# Autodesk Inventor assembly: uchwytDoSzyny
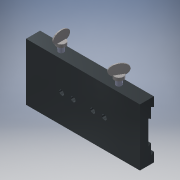
[picture p0: Inventor's stored thumbnail of the model, 180x180]
Saved by Autodesk Inventor 2019 (Build 230136000, 136)
## iProperties
Created: 2020-08-30
Part Number: uchwytDoSzyny
Document SubType Name: Assembly
Designer: estee
Author: estee
## Documents named in this file (3)
- C:\Users\estee\OneDrive\Pulpit\estere\1\MUM\najnowszyGIT\Mechanika\Moduł obrotu RET Estera\projejt\projejt\uchwytDoSzyny.iam
- C:\Users\estee\OneDrive\Pulpit\estere\1\MUM\nowygit\Mechanika\Moduł obrotu DEK Bartek\odBartka\Thumb Screw.ipt
- C:\Users\estee\OneDrive\Pulpit\estere\1\MUM\nowygit\Mechanika\Moduł obrotu DEK Bartek\odBartka\czescuchwytu.ipt
## Components (3 placed, 2 different names)
1. Thumb Screw:1 — Mate:2, Mate:3
2. Thumb Screw:2 — Mate:1, Mate:4
3. czescuchwytu:1 — Mate:1, Mate:2, Mate:3, Mate:4
## Relationships (4: Mate 4)
- Mate:1: Thumb Screw:2 ↔ czescuchwytu:1
- Mate:2: Thumb Screw:1 ↔ czescuchwytu:1
- Mate:3 (10 mm): Thumb Screw:1 ↔ czescuchwytu:1
- Mate:4 (10 mm): Thumb Screw:2 ↔ czescuchwytu:1
